# Autodesk Inventor assembly: PVZ3A
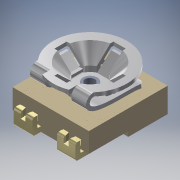
[picture p0: Inventor's stored thumbnail of the model, 180x180]
Saved by Autodesk Inventor 2016 (Build 200138000, 138)
## iProperties
Created: 2016-05-25
Part Number: PVZ3A
Document SubType Name: Assembly
Designer: Jonathan
Sending System: SOLIDWORKS 2016-2015258
MC: AMD64
MC_MODEL: Intel64 Family 6 Model 37 Stepping 1, GenuineIntel
OS: Windows_NT
FRU: Parasolid Version 28.0, build 174,  7- 3-2015
FORMAT: text
GUISE: transmit
FILE: 8D788D36-DBAC-42D3-9958-4A4E21655EB6.x_t
DATE: Wed May 25 10:02:46 2016
Author: Jonathan
## Documents named in this file (7)
- C:\Users\Jonathan\Documents\Projects\dynodePiShield\coincidenceCounter\cad\electronics\PVZ3A\PVZ3A.iam
- C:\Users\Jonathan\Documents\Projects\dynodePiShield\coincidenceCounter\cad\electronics\PVZ3A\User Library-PVZ3A_PVZ3A_base-1.ipt
- C:\Users\Jonathan\Documents\Projects\dynodePiShield\coincidenceCounter\cad\electronics\PVZ3A\User Library-PVZ3A_Pin1-1_2.ipt
- C:\Users\Jonathan\Documents\Projects\dynodePiShield\coincidenceCounter\cad\electronics\PVZ3A\User Library-PVZ3A_Pin2-1.ipt
- C:\Users\Jonathan\Documents\Projects\dynodePiShield\coincidenceCounter\cad\electronics\PVZ3A\User Library-PVZ3A_Pin2-2.ipt
- C:\Users\Jonathan\Documents\Projects\dynodePiShield\coincidenceCounter\cad\electronics\PVZ3A\User Library-PVZ3A_PVZ3A_res.ipt
- C:\Users\Jonathan\Documents\Projects\dynodePiShield\coincidenceCounter\cad\electronics\PVZ3A\User Library-PVZ3A_PVZ3A_con.ipt
## Components (6 placed, 6 different names)
1. User Library-PVZ3A_PVZ3A_base-1 — Mate:1, Mate:2, Angle:1, Mate:3, Mate:4, Mate:5, Mate:6, Mate:7, Mate:8, Mate:9, Mate:10
2. User Library-PVZ3A_Pin1-1_2 — Mate:4, Mate:5
3. User Library-PVZ3A_Pin2-1 — Mate:6, Mate:7
4. User Library-PVZ3A_Pin2-2 — Mate:8, Mate:9
5. User Library-PVZ3A_PVZ3A_res — Mate:1, Mate:2, Angle:1
6. User Library-PVZ3A_PVZ3A_con — Mate:3, Mate:10
## Relationships (11: Mate 10, Angle 1)
- Mate:1: User Library-PVZ3A_PVZ3A_base-1 ↔ User Library-PVZ3A_PVZ3A_res
- Mate:2: User Library-PVZ3A_PVZ3A_base-1 ↔ User Library-PVZ3A_PVZ3A_res
- Angle:1 (0 deg): User Library-PVZ3A_PVZ3A_base-1 ↔ User Library-PVZ3A_PVZ3A_res
- Mate:3: User Library-PVZ3A_PVZ3A_base-1 ↔ User Library-PVZ3A_PVZ3A_con
- Mate:4: User Library-PVZ3A_PVZ3A_base-1 ↔ User Library-PVZ3A_Pin1-1_2
- Mate:5: User Library-PVZ3A_PVZ3A_base-1 ↔ User Library-PVZ3A_Pin1-1_2
- Mate:6: User Library-PVZ3A_PVZ3A_base-1 ↔ User Library-PVZ3A_Pin2-1
- Mate:7: User Library-PVZ3A_PVZ3A_base-1 ↔ User Library-PVZ3A_Pin2-1
- Mate:8: User Library-PVZ3A_PVZ3A_base-1 ↔ User Library-PVZ3A_Pin2-2
- Mate:9: User Library-PVZ3A_PVZ3A_base-1 ↔ User Library-PVZ3A_Pin2-2
- Mate:10: User Library-PVZ3A_PVZ3A_base-1 ↔ User Library-PVZ3A_PVZ3A_con
